# Autodesk Inventor assembly: Bolt1
Saved by Autodesk Inventor 2015 (Build 190159000, 159)
## iProperties
Created: 2014-08-07
Part Number: Bolt1
Document SubType Name: Assembly
Designer: Patrick Camilleri
Author: Patrick Camilleri
## Documents named in this file (4)
- C:\Users\Patrick Camilleri\CAD\Test Box\Bolt1.iam
- C:\Users\Patrick Camilleri\Documents\Inventor\Content Center Files\R2015\en-US\GB_T 5782-2000\Bolt GB_T 5782 M8 x 70.ipt
- C:\Users\Patrick Camilleri\Documents\Inventor\Content Center Files\R2015\en-US\GB_T 6172.1-2000\Nut GB_T 6172.1 M8.ipt
- C:\Users\Patrick Camilleri\Documents\Inventor\Content Center Files\R2015\en-US\Washer GB_T 5652-1985\Washer GB_T 5652-1985 8.ipt
## Components (4 placed, 3 different names)
1. Bolt GB/T 5782-2000 M8x70:1
2. Nut GB/T 6172.1-2000 M8:1
3. Washer GB/T 5652-1985 8:1
4. Washer GB/T 5652-1985 8:2
## Relationships (2: WeldJoint 2)
- [WeldJoint]: Bolt GB/T 5782-2000 M8x70:1 ↔ Washer GB/T 5652-1985 8:2
- [WeldJoint]: Nut GB/T 6172.1-2000 M8:1 ↔ Washer GB/T 5652-1985 8:1
